# Autodesk Inventor assembly: gesamt
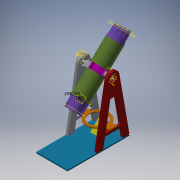
[picture p0: Inventor's stored thumbnail of the model, 180x180]
Saved by Autodesk Inventor 2017 (Build 210142000, 142)
## iProperties
Part Number: gesamt
Material: Generisch
Document SubType Name: Assembly
Designer: Fabio
Author: Fabio
## Documents named in this file (12)
- C:\Users\Fabio\dicer\inventor\gesamt.iam
- C:\Users\Fabio\dicer\inventor\grundplatte.ipt
- C:\Users\Fabio\dicer\inventor\halter_seite.ipt
- C:\Users\Fabio\dicer\inventor\spannring_achse.ipt
- C:\Users\Fabio\dicer\inventor\LED_Ring.ipt
- C:\Users\Fabio\dicer\inventor\spannring.ipt
- C:\Users\Fabio\dicer\inventor\cylinder.ipt
- C:\Users\Fabio\dicer\inventor\endkappen_V4.ipt
- C:\Users\Fabio\dicer\inventor\spiegelhalter.ipt
- C:\Users\Fabio\dicer\inventor\halter_seite_lager.ipt
- C:\Users\Fabio\dicer\inventor\spannring_achse_lager.ipt
- C:\Users\Fabio\dicer\inventor\endkappen_glashalter.ipt
## Components (13 placed, 11 different names)
1. grundplatte:1 — Passend:1, Passend:3, Passend:4, Passend:13, Einfügen:8, Einfügen:9
2. halter_seite:2 — Passend:1, Passend:3, Passend:4, Passend:14, Fluchtend:1
3. spannring_achse:2 — Passend:14, Fluchtend:1, Einfügen:10, Einfügen:11
4. LED_Ring:1 — Passend:18
5. spannring:1 — Einfügen:10, Einfügen:11
6. cylinder:1 — Einfügen:6, Einfügen:7, Passend:17
7. endkappen_V4:1 — Einfügen:6, Einfügen:14, Einfügen:15
8. endkappen_V4:2 — Einfügen:7
9. spiegelhalter:2 — Passend:13
10. halter_seite_lager:1 — Einfügen:8, Einfügen:9, Passend:15, Passend:16, Passend:18
11. spannring_achse_lager:1 — Passend:15, Passend:16, Einfügen:12, Einfügen:13
12. spannring:2 — Einfügen:12, Einfügen:13, Passend:17
13. endkappen_glashalter:1 — Einfügen:14, Einfügen:15
## Relationships (20: Insert 10, Mate 9, Flush 1)
- Passend:1 [Mate]: grundplatte:1 ↔ halter_seite:2
- Passend:3 [Mate]: grundplatte:1 ↔ halter_seite:2
- Passend:4 [Mate]: grundplatte:1 ↔ halter_seite:2
- Einfügen:6 [Insert]: cylinder:1 ↔ endkappen_V4:1
- Einfügen:7 [Insert]: cylinder:1 ↔ endkappen_V4:2
- Passend:13 [Mate]: grundplatte:1 ↔ spiegelhalter:2
- Einfügen:8 [Insert]: grundplatte:1 ↔ halter_seite_lager:1
- Einfügen:9 [Insert]: grundplatte:1 ↔ halter_seite_lager:1
- Passend:14 [Mate]: halter_seite:2 ↔ spannring_achse:2
- Fluchtend:1 [Flush]: halter_seite:2 ↔ spannring_achse:2
- Einfügen:10 [Insert]: spannring_achse:2 ↔ spannring:1
- Einfügen:11 [Insert]: spannring_achse:2 ↔ spannring:1
- Passend:15 [Mate]: halter_seite_lager:1 ↔ spannring_achse_lager:1
- Passend:16 [Mate]: halter_seite_lager:1 ↔ spannring_achse_lager:1
- Einfügen:12 [Insert]: spannring_achse_lager:1 ↔ spannring:2
- Einfügen:13 [Insert]: spannring_achse_lager:1 ↔ spannring:2
- Passend:17 [Mate]: cylinder:1 ↔ spannring:2
- Passend:18 [Mate]: LED_Ring:1 ↔ halter_seite_lager:1
- Einfügen:14 [Insert]: endkappen_V4:1 ↔ endkappen_glashalter:1
- Einfügen:15 [Insert]: endkappen_V4:1 ↔ endkappen_glashalter:1
